# Autodesk Inventor assembly: Smart-ControllerandBracket
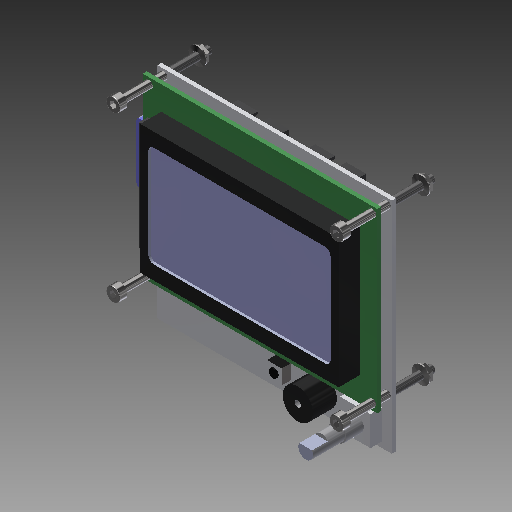
[picture p0: Inventor's stored thumbnail of the model, 512x512]
Saved by Autodesk Inventor 2017 (Build 210142000, 142)
## iProperties
Created: 2016-07-27
Part Number: Smart-ControllerandBracket
Document SubType Name: Assembly
Designer: User
Author: User
## Documents named in this file (5)
- C:\All INVENTOR\SL-Inventor\SL-Beast 3D Printer\Smart-ControllerandBracket.iam
- C:\All INVENTOR\SL-Inventor\SL-Beast 3D Printer\Full Graphic Smart Controller.ipt
- C:\All INVENTOR\SL-Inventor\SL-Beast 3D Printer\en-US\ANSI B18.3.1M(6)\ANSI B18.3.1M - M3x0.5 x 35(1).ipt
- C:\All INVENTOR\SL-Inventor\SL-Beast 3D Printer\en-US\JIS B 1251 C1 (1L 1H)\JIS B 1251  - 3 1L.ipt
- C:\All INVENTOR\SL-Inventor\SL-Beast 3D Printer\en-US\CSN EN 24 036\CSN EN 24 036 - M3.ipt
## Components (13 placed, 4 different names)
1. Full Graphic Smart Controller:1
2. Forged Socket Head Cap Screw - Metric M3x0.5 x 35:1
3. Forged Socket Head Cap Screw - Metric M3x0.5 x 35:2
4. JIS B 1251 Class 1 (1L/1H) 3 1L:1
5. JIS B 1251 Class 1 (1L/1H) 3 1L:2
6. CSN EN 24036 M3:1
7. CSN EN 24036 M3:2
8. Forged Socket Head Cap Screw - Metric M3x0.5 x 35:3
9. Forged Socket Head Cap Screw - Metric M3x0.5 x 35:4
10. JIS B 1251 Class 1 (1L/1H) 3 1L:3
11. JIS B 1251 Class 1 (1L/1H) 3 1L:4
12. CSN EN 24036 M3:3
13. CSN EN 24036 M3:4
## Relationships (8: Mate 8)
- [Mate]: Forged Socket Head Cap Screw - Metric M3x0.5 x 35:1 ↔ JIS B 1251 Class 1 (1L/1H) 3 1L:1
- [Mate]: Forged Socket Head Cap Screw - Metric M3x0.5 x 35:2 ↔ JIS B 1251 Class 1 (1L/1H) 3 1L:2
- [Mate]: Forged Socket Head Cap Screw - Metric M3x0.5 x 35:1 ↔ CSN EN 24036 M3:1
- [Mate]: Forged Socket Head Cap Screw - Metric M3x0.5 x 35:2 ↔ CSN EN 24036 M3:2
- [Mate]: Forged Socket Head Cap Screw - Metric M3x0.5 x 35:3 ↔ JIS B 1251 Class 1 (1L/1H) 3 1L:3
- [Mate]: Forged Socket Head Cap Screw - Metric M3x0.5 x 35:4 ↔ JIS B 1251 Class 1 (1L/1H) 3 1L:4
- [Mate]: Forged Socket Head Cap Screw - Metric M3x0.5 x 35:3 ↔ CSN EN 24036 M3:3
- [Mate]: Forged Socket Head Cap Screw - Metric M3x0.5 x 35:4 ↔ CSN EN 24036 M3:4
## Named parameters: d16_d22 = 0 mm, d18_d24 = 0 mm, d20_d26 = 0 mm
